# Autodesk Inventor assembly: Clamp(maxOpening40mm)-HumanBrainChunk
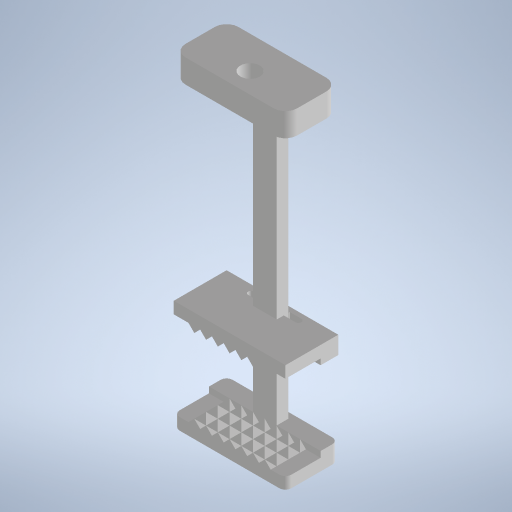
[picture p0: Inventor's stored thumbnail of the model, 512x512]
Saved by Autodesk Inventor 2023 (Build 270158000, 158)
## iProperties
Created: 2023-02-13
Part Number: Clamp(maxOpening40mm)-HumanBrainChunk
Document SubType Name: Assembly
Designer: nvladi
Author: nvladi
## Documents named in this file (3)
- C:\Users\Public\github\benchtop-hardware\Benchtop\custom-parts\sample_handling\assemblies\Clamp(maxOpening40mm)-HumanBrainChunk.iam
- C:\Users\Public\github\benchtop-hardware\Benchtop\custom-parts\sample_handling\sample-holders\Clamp-part1-Base9x19mm-maxSample40mm.ipt
- C:\Users\Public\github\benchtop-hardware\Benchtop\custom-parts\sample_handling\sample-holders\Clamp-part2(moving)-Base9x19mm_100912(01)_C.ipt
## Components (2 placed, 2 different names)
1. Clamp-part1-Base9x19mm-maxSample40mm:1 — Mate:1, Mate:2
2. Clamp-part2(moving)-Base9x19mm_100912(01)_C:1 — Mate:1, Mate:2
## Relationships (2: Mate 2)
- Mate:1: Clamp-part1-Base9x19mm-maxSample40mm:1 ↔ Clamp-part2(moving)-Base9x19mm_100912(01)_C:1
- Mate:2: Clamp-part1-Base9x19mm-maxSample40mm:1 ↔ Clamp-part2(moving)-Base9x19mm_100912(01)_C:1
